# Autodesk Inventor assembly: Button Fixture Assembly
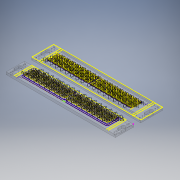
[picture p0: Inventor's stored thumbnail of the model, 180x180]
Saved by Autodesk Inventor 2018 (Build 220112000, 112)
## iProperties
Created: 2016-07-07
Part Number: Button Fixture Assembly
Document SubType Name: Assembly
Designer: Sam Clay
Author: Sam Clay
## Documents named in this file (3)
- Z:\enclosure\inventor\Button Fixture Assembly.iam
- Z:\enclosure\inventor\Button Fixture Base.ipt
- Z:\enclosure\inventor\Case Buttons CAM.ipt
## Components (65 placed, 2 different names)
1. Button Fixture Base:1 — Mate:7, Mate:8, Mate:9, Mate:10, Mate:11, Mate:12
2. Case Buttons CAM:9
3. Case Buttons CAM:10
4. Case Buttons CAM:11 — Mate:9
5. Case Buttons CAM:12
6. Case Buttons CAM:41
7. Case Buttons CAM:42
8. Case Buttons CAM:43
9. Case Buttons CAM:44
10. Case Buttons CAM:45 — Mate:7, Mate:8
11. Case Buttons CAM:46
12. Case Buttons CAM:47
13. Case Buttons CAM:48
14. Case Buttons CAM:49
15. Case Buttons CAM:50
16. Case Buttons CAM:51
17. Case Buttons CAM:52
18. Case Buttons CAM:25
19. Case Buttons CAM:26
20. Case Buttons CAM:27
21. Case Buttons CAM:28
22. Case Buttons CAM:53
23. Case Buttons CAM:54
24. Case Buttons CAM:55
25. Case Buttons CAM:87
26. Case Buttons CAM:57
27. Case Buttons CAM:58
28. Case Buttons CAM:59
29. Case Buttons CAM:60
30. Case Buttons CAM:61
31. Case Buttons CAM:62
32. Case Buttons CAM:63
33. Case Buttons CAM:86
34. Case Buttons CAM:17 — Mate:10, Mate:11, Mate:12
35. Case Buttons CAM:18
36. Case Buttons CAM:19
37. Case Buttons CAM:20
38. Case Buttons CAM:64
39. Case Buttons CAM:65
40. Case Buttons CAM:66
41. Case Buttons CAM:67
42. Case Buttons CAM:68
43. Case Buttons CAM:69
44. Case Buttons CAM:70
45. Case Buttons CAM:71
46. Case Buttons CAM:72
47. Case Buttons CAM:73
48. Case Buttons CAM:74
49. Case Buttons CAM:75
50. Case Buttons CAM:29
51. Case Buttons CAM:30
52. Case Buttons CAM:31
53. Case Buttons CAM:32
54. Case Buttons CAM:76
55. Case Buttons CAM:77
56. Case Buttons CAM:78
57. Case Buttons CAM:79
58. Case Buttons CAM:80
59. Case Buttons CAM:81
60. Case Buttons CAM:82
61. Case Buttons CAM:83
62. Case Buttons CAM:84
63. Case Buttons CAM:85
64. Case Buttons CAM:88
65. Case Buttons CAM:89
## Component patterns: (2 elements), (2 elements), (16 elements, first: Case Buttons CAM:9), Component Pattern 3:2 (16 elements), (16 elements, first: Case Buttons CAM:17), Component Pattern 4:2 (16 elements)
## Relationships (6: Mate 6)
- Mate:7 (0.7937 mm): Button Fixture Base:1 ↔ Case Buttons CAM:45
- Mate:8 (6.35 mm): Button Fixture Base:1 ↔ Case Buttons CAM:45
- Mate:9 (0.762 mm): Button Fixture Base:1 ↔ Case Buttons CAM:11
- Mate:10 (11.43 mm): Button Fixture Base:1 ↔ Case Buttons CAM:17
- Mate:11 (-25.4 mm): Button Fixture Base:1 ↔ Case Buttons CAM:17
- Mate:12 (-38.1 mm): Button Fixture Base:1 ↔ Case Buttons CAM:17
